# Autodesk Inventor assembly: BDinv
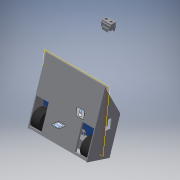
[picture p0: Inventor's stored thumbnail of the model, 180x180]
Saved by Autodesk Inventor 2017 (Build 210142000, 142)
## iProperties
Part Number: BDinv
Material: Ogólny
Document SubType Name: Assembly
Designer: Marek
Author: Marek
## Documents named in this file (10)
- D:\Studia\KoNaR\Biala-Dama\BDinv.iam
- D:\Studia\KoNaR\PCB.ipt
- D:\Studia\KoNaR\Materiały 2016\pololu_of.ipt
- D:\Studia\KoNaR\Materiały 2016\kolo_solar.ipt
- D:\Studia\KoNaR\Blacha wierzchnia.ipt
- D:\Studia\KoNaR\podstawa1.ipt
- D:\Studia\KoNaR\pług.ipt
- D:\Studia\KoNaR\Materiały 2016\mocowaniepololu.ipt
- D:\Studia\KoNaR\Materiały 2016\sharp.ipt
- D:\Studia\KoNaR\Materiały 2016\lipol.ipt
## Components (16 placed, 9 different names)
1. pololu_of:2 — Obrotowe:2, Sztywne:6, Zestawiający:8, Zestawiający:10, Sztywne:8
2. pololu_of:3 — Obrotowe:1, Obrotowe:3, Sztywne:7, Zestawiający:7, Zestawiający:11, Zestawiający:13
3. kolo_solar:1 — Obrotowe:1, Obrotowe:3, Styczny:1, Zestawiający:5
4. kolo_solar:2 — Obrotowe:2, Styczny:2, Zestawiający:6
5. Blacha wierzchnia:1 — Sztywne:5
6. podstawa1:1 — Sztywne:4, Zestawiający:1, Zestawiający:2, Zestawiający:3, Kąt:1, Zestawiający:4, Kąt:2
7. pług:1 — Sztywne:4, Sztywne:5, Zestawiający:12
8. PCB:1 — Równoległy:1, Sztywne:8, Zestawiający:14, Zestawiający:15, Zestawiający:16, Zestawiający:17, Zestawiający:18
9. mocowaniepololu:1 — Sztywne:7
10. mocowaniepololu:2 — Sztywne:6
11. sharp:1 — Zestawiający:14
12. sharp:2
13. sharp:3 — Zestawiający:16
14. sharp:4 — Zestawiający:17
15. sharp:5 — Zestawiający:15
16. lipol:1 — Zestawiający:18
## Relationships (31: Mate 18, WeldJoint 5, RevoluteJoint 3, Tangent 2, Angle 2, Flush 1)
- Obrotowe:1 [RevoluteJoint] (-1 mm): pololu_of:3 ↔ kolo_solar:1
- Obrotowe:2 [RevoluteJoint] (-1 mm): pololu_of:2 ↔ kolo_solar:2
- Sztywne:4 [WeldJoint]: podstawa1:1 ↔ pług:1
- Sztywne:5 [WeldJoint]: Blacha wierzchnia:1 ↔ pług:1
- Obrotowe:3 [RevoluteJoint] (-1 mm): pololu_of:3 ↔ kolo_solar:1
- Sztywne:6 [WeldJoint]: pololu_of:2 ↔ mocowaniepololu:2
- Sztywne:7 [WeldJoint]: pololu_of:3 ↔ mocowaniepololu:1
- Zestawiający:1 [Mate]: podstawa1:1
- Zestawiający:2 [Mate]: podstawa1:1
- Styczny:1 [Tangent]: kolo_solar:1
- Styczny:2 [Tangent]: kolo_solar:2
- Zestawiający:3 [Mate]: podstawa1:1
- Kąt:1 [Angle] (0 deg): podstawa1:1
- Zestawiający:4 [Mate]: podstawa1:1
- Kąt:2 [Angle] (0 deg): podstawa1:1
- Zestawiający:5 [Mate]: kolo_solar:1
- Zestawiający:6 [Mate]: kolo_solar:2
- Zestawiający:7 [Mate]: pololu_of:3
- Zestawiający:8 [Mate]: pololu_of:2
- Zestawiający:9 [Mate]
- Zestawiający:10 [Mate]: pololu_of:2
- Zestawiający:11 [Mate]: pololu_of:3
- Zestawiający:12 [Mate]: pług:1
- Zestawiający:13 [Mate]: pololu_of:3
- Równoległy:1 [Flush]: PCB:1
- Sztywne:8 [WeldJoint]: pololu_of:2 ↔ PCB:1
- Zestawiający:14 [Mate]: PCB:1 ↔ sharp:1
- Zestawiający:15 [Mate]: PCB:1 ↔ sharp:5
- Zestawiający:16 [Mate]: PCB:1 ↔ sharp:3
- Zestawiający:17 [Mate]: PCB:1 ↔ sharp:4
- Zestawiający:18 [Mate] (10 mm): PCB:1 ↔ lipol:1
